# Autodesk Inventor assembly: assembly
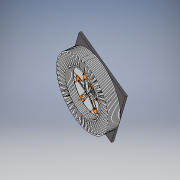
[picture p0: Inventor's stored thumbnail of the model, 180x180]
Saved by Autodesk Inventor 2018 (Build 220112000, 112)
## iProperties
Created: 2024-05-02
Part Number: assembly
Document SubType Name: Assembly
Designer: neo
Author: neo
## Documents named in this file (5)
- D:\projects\kreion\design1\3d\assembly.iam
- D:\projects\kreion\design1\3d\ring-holder.iam
- D:\projects\kreion\design1\3d\rotor-with-sliders.iam
- D:\projects\kreion\design1\3d\bottom-plate.ipt
- D:\projects\kreion\design1\3d\pleuel.ipt
## Components (9 placed, 4 different names)
1. ring-holder:1 [sub-assembly] — Insert:1
2. rotor-with-sliders:1 [sub-assembly] — Insert:1, Insert:2, Mate:1, Tangent:2, Tangent:3, Tangent:6, Tangent:8, Tangent:10, Tangent:12
3. bottom-plate:1 — Insert:2, Tangent:1, Tangent:4, Tangent:5, Tangent:7, Tangent:9, Tangent:11
4. pleuel:1 — Mate:1, Tangent:1, Tangent:2, Mate:2
5. pleuel:2 — Mate:2, Tangent:3, Tangent:4, Mate:3
6. pleuel:3 — Mate:3, Tangent:5, Tangent:6, Mate:4
7. pleuel:4 — Mate:4, Tangent:7, Tangent:8, Mate:5
8. pleuel:5 — Mate:5, Tangent:9, Tangent:10, Mate:6
9. pleuel:6 — Tangent:11, Mate:6, Tangent:12
## Relationships (20: Tangent 12, Mate 6, Insert 2)
- Insert:1 (-20 mm): ring-holder:1 ↔ rotor-with-sliders:1
- Insert:2: rotor-with-sliders:1 ↔ bottom-plate:1
- Mate:1: rotor-with-sliders:1 ↔ pleuel:1
- Tangent:1: bottom-plate:1 ↔ pleuel:1
- Tangent:2: rotor-with-sliders:1 ↔ pleuel:1
- Mate:2: pleuel:1 ↔ pleuel:2
- Tangent:3: rotor-with-sliders:1 ↔ pleuel:2
- Tangent:4: bottom-plate:1 ↔ pleuel:2
- Mate:3: pleuel:2 ↔ pleuel:3
- Tangent:5: bottom-plate:1 ↔ pleuel:3
- Tangent:6: rotor-with-sliders:1 ↔ pleuel:3
- Mate:4: pleuel:3 ↔ pleuel:4
- Tangent:7: bottom-plate:1 ↔ pleuel:4
- Tangent:8: rotor-with-sliders:1 ↔ pleuel:4
- Mate:5: pleuel:4 ↔ pleuel:5
- Tangent:9: bottom-plate:1 ↔ pleuel:5
- Tangent:10: rotor-with-sliders:1 ↔ pleuel:5
- Tangent:11: bottom-plate:1 ↔ pleuel:6
- Mate:6: pleuel:5 ↔ pleuel:6
- Tangent:12: rotor-with-sliders:1 ↔ pleuel:6
